# Autodesk Inventor assembly: Coverwithcameraholder
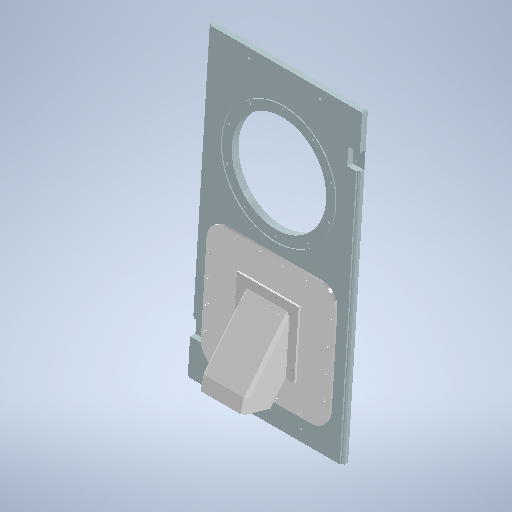
[picture p0: Inventor's stored thumbnail of the model, 512x512]
Saved by Autodesk Inventor 2025.2 (Build 292293000, 293)
## iProperties
Created: 2025-07-16
Part Number: Coverwithcameraholder
Document SubType Name: Assembly
Designer: mateo
Author: mateo
## Documents named in this file (7)
- C:\GitHub\In-situ-monitoring-of-powder-bed-fusion-additive-manufacturing\system_development\Damascus\hardware\Coverwithcameraholder.iam
- C:\GitHub\In-situ-monitoring-of-powder-bed-fusion-additive-manufacturing\system_development\Damascus\hardware\Xi 410 Camera.iam
- C:\GitHub\In-situ-monitoring-of-powder-bed-fusion-additive-manufacturing\system_development\Damascus\hardware\the big cover v1.ipt
- C:\GitHub\In-situ-monitoring-of-powder-bed-fusion-additive-manufacturing\system_development\Damascus\hardware\Reducer Plate.ipt
- C:\GitHub\In-situ-monitoring-of-powder-bed-fusion-additive-manufacturing\system_development\Mithril\v0.2\Hardware_design\flircamera+lens.ipt
- C:\GitHub\In-situ-monitoring-of-powder-bed-fusion-additive-manufacturing\system_development\Damascus\hardware\cameraholderbody v02.ipt
- C:\GitHub\In-situ-monitoring-of-powder-bed-fusion-additive-manufacturing\system_development\Damascus\hardware\cameraholderlid v02.ipt
## Components (6 placed, 6 different names)
1. Xi 410 Camera:1 [sub-assembly] — Insert:7
2. the big cover v1:1 — Insert:1
3. Reducer Plate:1 — Insert:1, Insert:5
4. flircamera+lens:1 — Insert:2, Insert:3
5. cameraholderbody v02:1 — Insert:2, Insert:3, Insert:5, Insert:6, Insert:7
6. cameraholderlid v02:1 — Insert:6
## Relationships (6: Insert 6)
- Insert:1: the big cover v1:1 ↔ Reducer Plate:1
- Insert:2: flircamera+lens:1 ↔ cameraholderbody v02:1
- Insert:3: flircamera+lens:1 ↔ cameraholderbody v02:1
- Insert:5: Reducer Plate:1 ↔ cameraholderbody v02:1
- Insert:6: cameraholderbody v02:1 ↔ cameraholderlid v02:1
- Insert:7: Xi 410 Camera:1 ↔ cameraholderbody v02:1
